# Autodesk Inventor assembly: Pen and Eraser Assembly
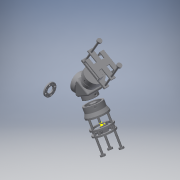
[picture p0: Inventor's stored thumbnail of the model, 180x180]
Saved by Autodesk Inventor 2019 (Build 230136000, 136)
## iProperties
Created: 2019-06-10
Part Number: Pen and Eraser Assembly
Document SubType Name: Assembly
Designer: Matthew XPS
Author: Matthew XPS
## Documents named in this file (10)
- G:\My Drive\Documents\Human Robot Interaction Lab\Projects\2019-06 Adept Viper Robot Arm\Pen  Holder\Pen and Eraser Assembly.iam
- G:\My Drive\Documents\Human Robot Interaction Lab\Projects\2019-06 Adept Viper Robot Arm\Pen  Holder\Clamp Plate.ipt
- G:\My Drive\Documents\Human Robot Interaction Lab\Projects\2019-06 Adept Viper Robot Arm\Pen  Holder\New Interface.ipt
- G:\My Drive\Documents\Human Robot Interaction Lab\Projects\2019-06 Adept Viper Robot Arm\Pen  Holder\Pen Main Piece.ipt
- G:\My Drive\Documents\Human Robot Interaction Lab\Projects\2019-06 Adept Viper Robot Arm\Pen  Holder\Robot Flange.ipt
- G:\My Drive\Documents\Human Robot Interaction Lab\Projects\2019-06 Adept Viper Robot Arm\Pen  Holder\6mm rod.ipt
- G:\My Drive\Documents\Human Robot Interaction Lab\Projects\2019-06 Adept Viper Robot Arm\Pen  Holder\6mm rod topper.ipt
- G:\My Drive\Documents\Human Robot Interaction Lab\Projects\2019-06 Adept Viper Robot Arm\Pen  Holder\Eraser + Pen Adapter.ipt
- G:\My Drive\Documents\Human Robot Interaction Lab\Projects\2019-06 Adept Viper Robot Arm\Pen  Holder\Eraser Interface.ipt
- G:\My Drive\Documents\Human Robot Interaction Lab\Projects\2019-06 Adept Viper Robot Arm\Pen  Holder\Eraser Holder.ipt
## Components (17 placed, 9 different names)
1. Clamp Plate:1 — Rotational:4
2. New Interface:1 — Rigid:2, Rotational:2, Rotational:3, Cylindrical:1
3. Pen Main Piece:1 — Mate:1, Mate:2, Mate:3, Rotational:4
4. Robot Flange:1
5. 6mm rod:1 — Rigid:2, Mate:1, Rigid:4
6. 6mm rod:2 — Rotational:2, Rigid:5, Mate:3
7. 6mm rod:3 — Rotational:3, Mate:2, Rigid:6
8. 6mm rod topper:1 — Rigid:4
9. 6mm rod topper:2 — Rigid:5
10. 6mm rod topper:3 — Rigid:6
11. Eraser + Pen Adapter:1 — Cylindrical:1, Mate:6
12. Eraser Interface:1 — Rigid:7, Rigid:8, Mate:6
13. 6mm rod:4 — Rigid:8, Mate:5, Rigid:9
14. 6mm rod:5 — Rigid:7, Mate:4, Rigid:10
15. Eraser Holder:1 — Mate:4, Mate:5
16. 6mm rod topper:4 — Rigid:9
17. 6mm rod topper:5 — Rigid:10
## Relationships (18: WeldJoint 8, Mate 6, RevoluteJoint 3, CylindricalJoint 1)
- Rigid:2 [WeldJoint]: New Interface:1 ↔ 6mm rod:1
- Rotational:2 [RevoluteJoint]: New Interface:1 ↔ 6mm rod:2
- Rotational:3 [RevoluteJoint]: New Interface:1 ↔ 6mm rod:3
- Mate:1: Pen Main Piece:1 ↔ 6mm rod:1
- Mate:2: Pen Main Piece:1 ↔ 6mm rod:3
- Rigid:4 [WeldJoint]: 6mm rod:1 ↔ 6mm rod topper:1
- Rigid:5 [WeldJoint]: 6mm rod:2 ↔ 6mm rod topper:2
- Rigid:6 [WeldJoint]: 6mm rod:3 ↔ 6mm rod topper:3
- Mate:3: Pen Main Piece:1 ↔ 6mm rod:2
- Cylindrical:1: New Interface:1 ↔ Eraser + Pen Adapter:1
- Rigid:7 [WeldJoint]: Eraser Interface:1 ↔ 6mm rod:5
- Rigid:8 [WeldJoint]: Eraser Interface:1 ↔ 6mm rod:4
- Mate:4: 6mm rod:5 ↔ Eraser Holder:1
- Mate:5: 6mm rod:4 ↔ Eraser Holder:1
- Mate:6: Eraser + Pen Adapter:1 ↔ Eraser Interface:1
- Rotational:4 [RevoluteJoint]: Clamp Plate:1 ↔ Pen Main Piece:1
- Rigid:9 [WeldJoint]: 6mm rod:4 ↔ 6mm rod topper:4
- Rigid:10 [WeldJoint]: 6mm rod:5 ↔ 6mm rod topper:5
